# Autodesk Inventor assembly: Sec_SecondStage_Enclosure
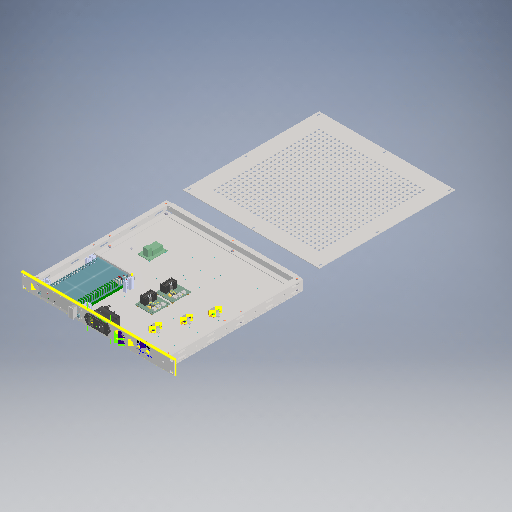
[picture p0: Inventor's stored thumbnail of the model, 512x512]
Saved by Autodesk Inventor 2025.2 (Build 292293000, 293)
## iProperties
Created: 2014-04-08
Part Number: Sec_SecondStage_Enclosure
Document SubType Name: Assembly
Designer: alexanderpollak
Sending System: Autodesk Inventor 2012
Preprocessor: Autodesk Inventor 2012
Title: Z:\Eng\Products\Research and Development\PENDING TBC\GDI VD4001\VD4001-00-0117.stp
Author: DonFlagin
## Documents named in this file (26)
- C:\Users\PaulLinke\Documents\Inventor\MyLibrary\Assemblies\RF-Assemblies\SEC_SecondStage_Enclosure\Sec_SecondStage_Enclosure.iam
- Sec_SecondStage_Enclosure.iam
- C:\Users\PaulLinke\Documents\Inventor\MyLibrary\Assemblies\RF-Assemblies\ATA_SNAP_Enclosure\VC4084-00-0017.iam
- C:\Users\PaulLinke\Documents\Inventor\MyLibrary\Assemblies\RF-Assemblies\ATA_SNAP_Enclosure\VC4027-00-0017.ipt
- C:\Users\PaulLinke\Documents\Inventor\MyLibrary\Assemblies\RF-Assemblies\ATA_SNAP_Enclosure\HA2137-06-4009.ipt
- C:\Users\PaulLinke\Documents\Inventor\MyLibrary\Assemblies\RF-Assemblies\ATA_SNAP_Enclosure\VC4039-00-0001.ipt
- C:\Users\PaulLinke\Documents\Inventor\MyLibrary\Assemblies\RF-Assemblies\ATA_SNAP_Enclosure\HA2112-06-5010.ipt
- C:\Users\PaulLinke\Documents\Inventor\MyLibrary\Assemblies\RF-Assemblies\ATA_SNAP_Enclosure\HA2350-06-1007.ipt
- C:\Users\PaulLinke\Documents\Inventor\MyLibrary\Assemblies\RF-Assemblies\ATA_SNAP_Enclosure\VC4084-00-0018.ipt
- C:\Users\PaulLinke\Documents\Inventor\MyLibrary\Assemblies\MISC\AC-Inlet\35718.iam
- C:\Users\PaulLinke\Documents\Inventor\MyLibrary\Assemblies\MISC\Max-Power-6HP\13100151.iam
- C:\Users\PaulLinke\Documents\Inventor\MyLibrary\Parts\MISC\SchroffThreadedInlay_30mm.ipt
- C:\Users\PaulLinke\Documents\Inventor\MyLibrary\Parts\MISC\SchroffRailNoExtrusion_30mm_Left.ipt
- C:\Users\PaulLinke\Documents\Inventor\MyLibrary\Parts\MISC\SchroffRailNoExtrusion_30mm_Right.ipt
- C:\Users\PaulLinke\Documents\Inventor\MyLibrary\Assemblies\RF-Assemblies\Mini-Circuits_BIAS-TEE_ZX85-12G-S+.iam
- C:\Users\PaulLinke\Documents\Inventor\MyLibrary\Assemblies\RF-Assemblies\Mini-Circuits_LNAmp_ZX60-14LN-S+.iam
- C:\Users\PaulLinke\Documents\Inventor\MyLibrary\Parts\MISC\Hex_standoff_M2.5_5mm_noPole.ipt
- C:\Users\PaulLinke\Documents\Inventor\MyLibrary\Parts\RF-Parts\Voltage_Regulator_for_ZX60-14LN-S+\Voltage_Regulator_for_ZX60-14LN-S+\Voltage_Regulator_for_ZX60-14LN-S+.iam
- C:\Users\PaulLinke\Documents\Inventor\MyLibrary\Assemblies\MISC\FlatLED_6mm.iam
- C:\Users\PaulLinke\Documents\Inventor\MyLibrary\Parts\RF-Parts\SMA_Feedthrough.ipt
- C:\Users\PaulLinke\Documents\Inventor\MyLibrary\Assemblies\RF-Assemblies\SEC_SecondStage_Enclosure\CaseScrew.ipt
- C:\Users\PaulLinke\Documents\Inventor\MyLibrary\Parts\MISC\DIN 660 - A 6 x 12 x 0.001.ipt
- C:\Users\PaulLinke\Documents\Inventor\Content Center Files\R2025\en-US\AS 1427(07)\AS 1427 - M3 x 5(6) II.ipt
- C:\Users\PaulLinke\Documents\Inventor\Content Center Files\R2025\en-US\BS 4183(2)\BS 4183 - M2.5 x 4(1) I.ipt
- C:\Users\PaulLinke\Documents\Inventor\MyLibrary\Parts\MISC\Schroff_Back_Stabilizer.ipt
- C:\Users\PaulLinke\Documents\Inventor\MyLibrary\Parts\MISC\NAS_Splitter_PCB.ipt
## Components (67 placed, 25 different names)
1. 1UCaseFrame:1 [sub-assembly] — Mate:1, Mate:2, Flush:1, Mate:4, Flush:2, Flush:5, Flush:6, Mate:26, Mate:28, Mate:29, Mate:30, Mate:31, Mate:32, Mate:33, Mate:35, Mate:37, Mate:38, Mate:39, Mate:40
2. TopPlate:1 — Mate:1, Flush:2
3. CaseScrew:1 — Mate:33, Mate:40, Mate:41
4. CaseScrew:2 — Mate:31, Mate:38, Mate:43
5. CaseScrew:3 — Mate:32, Mate:39, Mate:42
6. CaseScrew:4 — Mate:30, Mate:37, Mate:44
7. CaseScrew:5 — Mate:26, Mate:27
8. CaseScrew:6 — Mate:29, Mate:35, Mate:36
9. CaseScrew:7 — Mate:28, Mate:34
10. FrontPanel:1 — Mate:3, Mate:4, Flush:5, Flush:6, Insert:1, Flush:7, Mate:5, Mate:9, Mate:13, Mate:17, Mate:21, Mate:45, Mate:46, Mate:92, Mate:93, Mate:94, Mate:95, Mate:115, Mate:116, Mate:123, Mate:124, Mate:125, Mate:126
11. FrontPanelScrew:1 — Mate:46
12. FrontPanelScrew:2 — Mate:45
13. FrontPanelNut:1
14. FrontPanelNut:2
15. BottomPlate:1 — Mate:2, Mate:3, Flush:1, Mate:8, Mate:12, Mate:16, Mate:20, Mate:27, Mate:34, Mate:36, Mate:41, Mate:42, Mate:43, Mate:44, Mate:75, Mate:76, Mate:96, Mate:97, Mate:100, Mate:101, Mate:102, Mate:103, Mate:104, Mate:105, Mate:106, Mate:107, Mate:108, Mate:109, Mate:110, Mate:111, Mate:132, Mate:133, Mate:134
16. ACInlet:1 [sub-assembly] — Insert:1, Mate:121, Mate:122
17. PSU:1 [sub-assembly] — Flush:7, Mate:5, Mate:22, Mate:23
18. SchroffThreadedInlay_25mm:1 — Mate:6, Mate:7, Mate:23
19. SchroffThreadedInlay_25mm:3 — Mate:18, Mate:19, Mate:22
20. SchroffRailNoExtrusion_30mm_Left:3 — Mate:18, Mate:19, Mate:20, Mate:21, Mate:24, Flush:8, Mate:98
21. SchroffRailNoExtrusion_30mm_Left:4 — Mate:12, Mate:13, Mate:25
22. SchroffRailNoExtrusion_30mm_Right:2 — Mate:16, Mate:17, Mate:24
23. SchroffRailNoExtrusion_30mm_Right:3 — Mate:6, Mate:7, Mate:8, Mate:9, Mate:25, Flush:9, Mate:99
24. Mini-Circuits_BIAS-TEE_ZX85-12G-S+:1 [sub-assembly]
25. Voltage_Regulator_for_ZX60-14LN-S+:1 [sub-assembly] — Mate:63, Mate:64, Mate:65, Mate:67
26. Voltage_Regulator_for_ZX60-14LN-S+:2 [sub-assembly] — Mate:59, Mate:66, Mate:69, Mate:70
27. AS 1110 - Metric M2.5 x 6:12 — Mate:67
28. AS 1110 - Metric M2.5 x 6:13 — Mate:59
29. AS 1110 - Metric M2.5 x 6:16 — Mate:64, Mate:76
30. AS 1110 - Metric M2.5 x 6:17 — Mate:66
31. AS 1110 - Metric M2.5 x 6:19 — Mate:69
32. AS 1110 - Metric M2.5 x 6:20 — Mate:63
33. AS 1110 - Metric M2.5 x 6:21 — Mate:70, Mate:75
34. AS 1110 - Metric M2.5 x 6:22 — Mate:65
35. Mini-Circuits_LNAmp_ZX60-14LN-S+:2 [sub-assembly]
36. Mini-Circuits_BIAS-TEE_ZX85-12G-S+:3 [sub-assembly]
37. FlatLED_6mm:1 [sub-assembly] — Mate:92
38. FlatLED_6mm:2 [sub-assembly] — Mate:93
39. SMA_Feedthrough:1 — Mate:94
40. SMA_Feedthrough:2 — Mate:95
41. SchroffRailNoExtrusion_30mm_Right:4 — Mate:97, Flush:8, Mate:98, Mate:128, Mate:129
42. SchroffRailNoExtrusion_30mm_Left:5 — Mate:96, Flush:9, Mate:99, Mate:130, Mate:131
43. HA2137-06-4009:8 — Mate:101
44. HA2137-06-4009:9 — Mate:100
45. HA2137-06-4009:10 — Mate:111
46. HA2137-06-4009:11 — Mate:108
47. HA2137-06-4009:12 — Mate:109
48. HA2137-06-4009:13 — Mate:110
49. HA2137-06-4009:14 — Mate:107
50. HA2137-06-4009:15 — Mate:106
51. HA2137-06-4009:16 — Mate:104
52. HA2137-06-4009:17 — Mate:105
53. HA2137-06-4009:18 — Mate:103
54. HA2137-06-4009:19 — Mate:102
55. CaseScrew:1 — Mate:132
56. DIN 660 - A 6 x 12 x 0.001:1 — Mate:116
57. DIN 660 - A 6 x 12 x 0.001:2 — Mate:115
58. AS 1427 Z - Metric M3 x 5:1 — Mate:121
59. AS 1427 Z - Metric M3 x 5:2 — Mate:122
60. BS 4183 Cross Recessed Flat Countersunk Head Machine Screw - Metric M2.5 x 4:1 — Mate:123
61. BS 4183 Cross Recessed Flat Countersunk Head Machine Screw - Metric M2.5 x 4:2 — Mate:124
62. BS 4183 Cross Recessed Flat Countersunk Head Machine Screw - Metric M2.5 x 4:3 — Mate:125
63. BS 4183 Cross Recessed Flat Countersunk Head Machine Screw - Metric M2.5 x 4:4 — Mate:126
64. SchroffThreadedInlay_30mm:4 — Mate:130, Mate:131, Insert:3
65. SchroffThreadedInlay_30mm:5 — Mate:128, Mate:129, Insert:2
66. Schroff_Back_Stabilizer:1 — Insert:2, Insert:3
67. NAS_Splitter_PCB:1 — Mate:133, Mate:134
## Relationships (97: Mate 87, Flush 7, Insert 3)
- Mate:1: 1UCaseFrame:1 ↔ TopPlate:1
- Mate:2: 1UCaseFrame:1 ↔ BottomPlate:1
- Mate:3: FrontPanel:1 ↔ BottomPlate:1
- Flush:1 (-0.762 mm): 1UCaseFrame:1 ↔ BottomPlate:1
- Mate:4: 1UCaseFrame:1 ↔ FrontPanel:1
- Flush:2 (0.762 mm): 1UCaseFrame:1 ↔ TopPlate:1
- Flush:5 (-25.3873 mm): 1UCaseFrame:1 ↔ FrontPanel:1
- Flush:6 (5.969 mm): 1UCaseFrame:1 ↔ FrontPanel:1
- Insert:1: FrontPanel:1 ↔ ACInlet:1
- Flush:7: FrontPanel:1 ↔ PSU:1
- Mate:5 (0.05 mm): FrontPanel:1 ↔ PSU:1
- Mate:6: SchroffThreadedInlay_25mm:1 ↔ SchroffRailNoExtrusion_30mm_Right:3
- Mate:7 (0.125 mm): SchroffThreadedInlay_25mm:1 ↔ SchroffRailNoExtrusion_30mm_Right:3
- Mate:8: BottomPlate:1 ↔ SchroffRailNoExtrusion_30mm_Right:3
- Mate:9: FrontPanel:1 ↔ SchroffRailNoExtrusion_30mm_Right:3
- Mate:12: BottomPlate:1 ↔ SchroffRailNoExtrusion_30mm_Left:4
- Mate:13: FrontPanel:1 ↔ SchroffRailNoExtrusion_30mm_Left:4
- Mate:16: BottomPlate:1 ↔ SchroffRailNoExtrusion_30mm_Right:2
- Mate:17: FrontPanel:1 ↔ SchroffRailNoExtrusion_30mm_Right:2
- Mate:18: SchroffThreadedInlay_25mm:3 ↔ SchroffRailNoExtrusion_30mm_Left:3
- Mate:19 (0.125 mm): SchroffThreadedInlay_25mm:3 ↔ SchroffRailNoExtrusion_30mm_Left:3
- Mate:20: BottomPlate:1 ↔ SchroffRailNoExtrusion_30mm_Left:3
- Mate:21: FrontPanel:1 ↔ SchroffRailNoExtrusion_30mm_Left:3
- Mate:22: PSU:1 ↔ SchroffThreadedInlay_25mm:3
- Mate:23: PSU:1 ↔ SchroffThreadedInlay_25mm:1
- Mate:24: SchroffRailNoExtrusion_30mm_Left:3 ↔ SchroffRailNoExtrusion_30mm_Right:2
- Mate:25: SchroffRailNoExtrusion_30mm_Left:4 ↔ SchroffRailNoExtrusion_30mm_Right:3
- Mate:26: 1UCaseFrame:1 ↔ CaseScrew:5
- Mate:27: CaseScrew:5 ↔ BottomPlate:1
- Mate:28: 1UCaseFrame:1 ↔ CaseScrew:7
- Mate:29: 1UCaseFrame:1 ↔ CaseScrew:6
- Mate:30: 1UCaseFrame:1 ↔ CaseScrew:4
- Mate:31: 1UCaseFrame:1 ↔ CaseScrew:2
- Mate:32: 1UCaseFrame:1 ↔ CaseScrew:3
- Mate:33: 1UCaseFrame:1 ↔ CaseScrew:1
- Mate:34: CaseScrew:7 ↔ BottomPlate:1
- Mate:35: 1UCaseFrame:1 ↔ CaseScrew:6
- Mate:36: CaseScrew:6 ↔ BottomPlate:1
- Mate:37: 1UCaseFrame:1 ↔ CaseScrew:4
- Mate:38: 1UCaseFrame:1 ↔ CaseScrew:2
- Mate:39: 1UCaseFrame:1 ↔ CaseScrew:3
- Mate:40: 1UCaseFrame:1 ↔ CaseScrew:1
- Mate:41: CaseScrew:1 ↔ BottomPlate:1
- Mate:42: CaseScrew:3 ↔ BottomPlate:1
- Mate:43: CaseScrew:2 ↔ BottomPlate:1
- Mate:44: CaseScrew:4 ↔ BottomPlate:1
- Mate:45: FrontPanel:1 ↔ FrontPanelScrew:2
- Mate:46: FrontPanel:1 ↔ FrontPanelScrew:1
- Mate:59: Voltage_Regulator_for_ZX60-14LN-S+:2 ↔ AS 1110 - Metric M2.5 x 6:13
- Mate:63: Voltage_Regulator_for_ZX60-14LN-S+:1 ↔ AS 1110 - Metric M2.5 x 6:20
- Mate:64: Voltage_Regulator_for_ZX60-14LN-S+:1 ↔ AS 1110 - Metric M2.5 x 6:16
- Mate:65: Voltage_Regulator_for_ZX60-14LN-S+:1 ↔ AS 1110 - Metric M2.5 x 6:22
- Mate:66: Voltage_Regulator_for_ZX60-14LN-S+:2 ↔ AS 1110 - Metric M2.5 x 6:17
- Mate:67: Voltage_Regulator_for_ZX60-14LN-S+:1 ↔ AS 1110 - Metric M2.5 x 6:12
- Mate:69: Voltage_Regulator_for_ZX60-14LN-S+:2 ↔ AS 1110 - Metric M2.5 x 6:19
- Mate:70: Voltage_Regulator_for_ZX60-14LN-S+:2 ↔ AS 1110 - Metric M2.5 x 6:21
- Mate:75: BottomPlate:1 ↔ AS 1110 - Metric M2.5 x 6:21
- Mate:76: BottomPlate:1 ↔ AS 1110 - Metric M2.5 x 6:16
- Mate:92: FrontPanel:1 ↔ FlatLED_6mm:1
- Mate:93: FrontPanel:1 ↔ FlatLED_6mm:2
- Mate:94: FrontPanel:1 ↔ SMA_Feedthrough:1
- Mate:95: FrontPanel:1 ↔ SMA_Feedthrough:2
- Mate:96: BottomPlate:1 ↔ SchroffRailNoExtrusion_30mm_Left:5
- Mate:97: BottomPlate:1 ↔ SchroffRailNoExtrusion_30mm_Right:4
- Flush:8: SchroffRailNoExtrusion_30mm_Left:3 ↔ SchroffRailNoExtrusion_30mm_Right:4
- Flush:9: SchroffRailNoExtrusion_30mm_Right:3 ↔ SchroffRailNoExtrusion_30mm_Left:5
- Mate:98 (114 mm): SchroffRailNoExtrusion_30mm_Left:3 ↔ SchroffRailNoExtrusion_30mm_Right:4
- Mate:99 (114 mm): SchroffRailNoExtrusion_30mm_Right:3 ↔ SchroffRailNoExtrusion_30mm_Left:5
- Mate:100: BottomPlate:1 ↔ HA2137-06-4009:9
- Mate:101: BottomPlate:1 ↔ HA2137-06-4009:8
- Mate:102: BottomPlate:1 ↔ HA2137-06-4009:19
- Mate:103: BottomPlate:1 ↔ HA2137-06-4009:18
- Mate:104: BottomPlate:1 ↔ HA2137-06-4009:16
- Mate:105: BottomPlate:1 ↔ HA2137-06-4009:17
- Mate:106: BottomPlate:1 ↔ HA2137-06-4009:15
- Mate:107: BottomPlate:1 ↔ HA2137-06-4009:14
- Mate:108: BottomPlate:1 ↔ HA2137-06-4009:11
- Mate:109: BottomPlate:1 ↔ HA2137-06-4009:12
- Mate:110: BottomPlate:1 ↔ HA2137-06-4009:13
- Mate:111: BottomPlate:1 ↔ HA2137-06-4009:10
- Mate:115: FrontPanel:1 ↔ DIN 660 - A 6 x 12 x 0.001:2
- Mate:116: FrontPanel:1 ↔ DIN 660 - A 6 x 12 x 0.001:1
- Mate:121: ACInlet:1 ↔ AS 1427 Z - Metric M3 x 5:1
- Mate:122: ACInlet:1 ↔ AS 1427 Z - Metric M3 x 5:2
- Mate:123: FrontPanel:1 ↔ BS 4183 Cross Recessed Flat Countersunk Head Machine Screw - Metric M2.5 x 4:1
- Mate:124: FrontPanel:1 ↔ BS 4183 Cross Recessed Flat Countersunk Head Machine Screw - Metric M2.5 x 4:2
- Mate:125: FrontPanel:1 ↔ BS 4183 Cross Recessed Flat Countersunk Head Machine Screw - Metric M2.5 x 4:3
- Mate:126: FrontPanel:1 ↔ BS 4183 Cross Recessed Flat Countersunk Head Machine Screw - Metric M2.5 x 4:4
- Mate:128 (0.125 mm): SchroffRailNoExtrusion_30mm_Right:4 ↔ SchroffThreadedInlay_30mm:5
- Mate:129: SchroffRailNoExtrusion_30mm_Right:4 ↔ SchroffThreadedInlay_30mm:5
- Mate:130: SchroffRailNoExtrusion_30mm_Left:5 ↔ SchroffThreadedInlay_30mm:4
- Mate:131 (0.125 mm): SchroffRailNoExtrusion_30mm_Left:5 ↔ SchroffThreadedInlay_30mm:4
- Insert:2 (2.2 mm): SchroffThreadedInlay_30mm:5 ↔ Schroff_Back_Stabilizer:1
- Insert:3 (2.2 mm): SchroffThreadedInlay_30mm:4 ↔ Schroff_Back_Stabilizer:1
- Mate:132: BottomPlate:1 ↔ CaseScrew:1
- Mate:133 (4 mm): BottomPlate:1 ↔ NAS_Splitter_PCB:1
- Mate:134: BottomPlate:1 ↔ NAS_Splitter_PCB:1
